# Autodesk Inventor assembly: ASY NDM 11.050 перегородка рама 2 вертикал
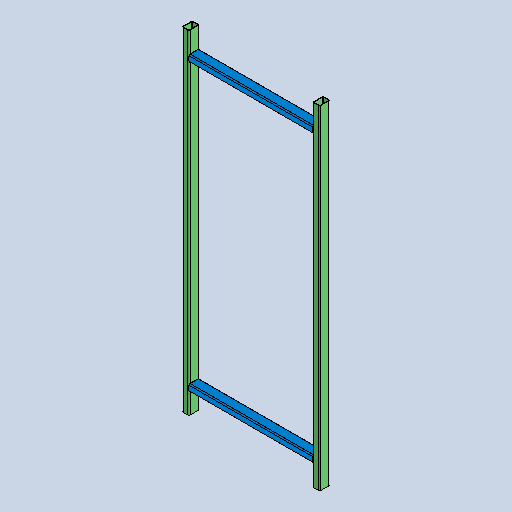
[picture p0: Inventor's stored thumbnail of the model, 512x512]
Saved by Autodesk Inventor 2025 (Build 290162010, 162A)
## iProperties
Created: 2024-08-12
Part Number: ASY NDM 11.050 перегородка рама 2 вертикал
Document SubType Name: Assembly
Designer: admin
_SolveAssemblyDoc: Frame Generator Solve Assembly
_Version: 25.0.0
Author: admin
## Documents named in this file (3)
- C:\Users\admin\YandexDisk-badmisterfox\домашниий пк\Inventor\BSH_Beshkino_bio_tank\лестница\Перегородка\ASY NDM 11.050 перегородка рама 2 вертикал.iam
- C:\Users\admin\YandexDisk-badmisterfox\домашниий пк\Inventor\BSH_Beshkino_bio_tank\лестница\Перегородка\NDM 11.042 рама 2 вертикал угол.ipt
- C:\Users\admin\YandexDisk-badmisterfox\домашниий пк\Inventor\BSH_Beshkino_bio_tank\лестница\Перегородка\ASY NDM 11.050 перегородка рама 2 вертикал\Frame\Frame 1723530770913.iam
## Components (2 placed, 2 different names)
1. NDM 11.042 рама 2 вертикал угол:1 — Mate:1, Mate:2, Flush:1
2. Frame 1723530770913:1 [sub-assembly]
## Relationships (3: Mate 2, Flush 1)
- Mate:1: NDM 11.042 рама 2 вертикал угол:1
- Mate:2: NDM 11.042 рама 2 вертикал угол:1
- Flush:1: NDM 11.042 рама 2 вертикал угол:1
